# Autodesk Inventor assembly: Shooter Assembly v2
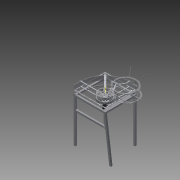
[picture p0: Inventor's stored thumbnail of the model, 180x180]
Saved by Autodesk Inventor 2013 (Build 170138000, 138)
## iProperties
Created: 2013-01-15
Part Number: Shooter Assembly v2
Document SubType Name: Assembly
Designer: actoennies
Mass: 7800.39 g
Surface Area: 25298.1 cm^2
Volume: 4142.24 cm^3
Density: 1.88313 g/cm^3
Author: actoennies
## Documents named in this file (24)
- C:\Users\Moses\Documents\GitHub\frc2013CAD\Launcher\Shooter\Shooter Assembly v2.iam
- C:\Users\Moses\Documents\GitHub\frc2013CAD\Launcher\Shooter\Bearing Mount v1.ipt
- C:\Users\Moses\Documents\GitHub\frc2013CAD\Launcher\Shooter\Outer Rail v1.ipt
- C:\Users\Moses\Documents\GitHub\frc2013CAD\Launcher\Shooter\Runner Rails v2.ipt
- C:\Users\Moses\Documents\GitHub\frc2013CAD\Launcher\Other\8 Plaction Wheel.iam
- C:\Users\Moses\Documents\GitHub\frc2013CAD\Launcher\Shooter\Hub v1.ipt
- C:\Users\Moses\Documents\GitHub\frc2013CAD\Launcher\Shooter\Bearing.ipt
- C:\Users\Moses\Documents\GitHub\frc2013CAD\Launcher\Shooter\Shaft.ipt
- C:\Users\Moses\Documents\GitHub\frc2013CAD\Launcher\Parts\Imported Components\Toughbox Nano 500 key\2mmx2mmx10mm_key.ipt
- C:\Users\Moses\Documents\GitHub\frc2013CAD\Launcher\Shooter\CIM Assembly.iam
- C:\Users\Moses\Documents\GitHub\frc2013CAD\Launcher\Shooter\Flywheel Assembly.iam
- C:\Users\Moses\Documents\GitHub\frc2013CAD\Launcher\Shooter\Shooter Mounter.ipt
- C:\Users\Moses\Documents\GitHub\frc2013CAD\Launcher\Shooter\Bearing Mount 2 v1.ipt
- C:\Users\Moses\Documents\GitHub\frc2013CAD\Launcher\Shooter\Shorter Shaft.ipt
- C:\Users\Moses\Documents\GitHub\frc2013CAD\Launcher\Shooter\Spacer Rube.ipt
- C:\Users\Moses\Documents\GitHub\frc2013CAD\Launcher\Shooter\Tower Angled Mount.ipt
- C:\Users\Moses\Documents\GitHub\frc2013CAD\Launcher\Shooter\Edge Mount.ipt
- C:\Users\Moses\Documents\GitHub\frc2013CAD\Launcher\Shooter\Tower Corner Mount.ipt
- C:\Users\Moses\Documents\GitHub\frc2013CAD\Launcher\Shooter\Square Tube.ipt
- C:\Users\Moses\Documents\GitHub\frc2013CAD\Launcher\Shooter\Flange Bearing Mount Tower.ipt
- C:\Users\Moses\Documents\GitHub\frc2013CAD\Launcher\Shooter\Flange Bearing Mount Tower Mirror.ipt
- C:\Users\Moses\Documents\GitHub\frc2013CAD\Launcher\Shooter\Bearing Mount Top.ipt
- C:\Users\Moses\Documents\GitHub\frc2013CAD\Launcher\Shooter\Square Motor Mount.ipt
- C:\Users\Moses\Documents\GitHub\frc2013CAD\Launcher\Hopper\HopperAssembly42inch_v5.iam
## Components (36 placed, 23 different names)
1. Bearing Mount v1:1 — Insert:12, Insert:13, Insert:14, Insert:15, Insert:19, Angle:1, Insert:26, Insert:27
2. Outer Rail v1:1 — Insert:12, Insert:13, Insert:47, Insert:48, Flush:21
3. Runner Rails v2:1 — Insert:14, Insert:15, Mate:42
4. 8 Plaction Wheel:1 [sub-assembly] — Insert:21, Insert:22, Rotation:1
5. Hub v1:1 — Insert:21, Flush:3, Insert:23
6. Hub v1:2 — Insert:22, Flush:3, Rotation:1, Mate:6
7. Bearing:1 — Mate:3, Insert:49
8. Bearing:2 — Insert:19, Mate:1, Mate:2, Insert:23
9. Shaft:1 — Mate:1, Mate:2, Mate:3, Flush:4, Mate:4, Mate:5, Mate:6, Mate:7, Mate:8, Flush:5
10. 2mmx2mmx10mm_key:1
11. CIM Assembly:1 [sub-assembly] — Flush:4, Mate:4, Mate:5, Angle:1, Mate:9, Mate:10, Mate:11
12. Flywheel Assembly:1 [sub-assembly] — Mate:7, Mate:8, Flush:5, Mate:39
13. Shooter Mounter:1 — Insert:26, Insert:27, Insert:34, Flush:11, Mate:10, Mate:11, Insert:35, Insert:36, Insert:37, Insert:38, Flush:19
14. Spacer Rube:1 — Insert:34, Flush:11
15. Bearing Mount 2 v1:1 — Insert:37, Insert:38, Insert:40
16. Bearing Mount 2 v1:2 — Insert:35, Insert:36, Insert:39
17. Bearing:3 — Insert:40, Flush:13, Mate:14, Mate:15
18. Bearing:4 — Insert:39, Flush:12, Mate:12, Mate:13, Mate:36
19. Shorter Shaft:1 — Flush:12, Mate:12, Mate:13, Mate:37
20. Shorter Shaft:2 — Flush:13, Mate:14, Mate:15, Mate:38
21. Tower Angled Mount:1 — Mate:34, Flush:18, Mate:35, Mate:40, Flush:20
22. Edge Mount:1 — Mate:18, Flush:15, Mate:19, Mate:20, Mate:41
23. Tower Corner Mount:1 — Mate:16, Flush:14, Mate:17
24. Edge Mount:2 — Mate:24, Mate:25, Flush:17, Mate:26, Mate:28
25. Square Tube:1 — Mate:20, Mate:21, Mate:33, Mate:34, Flush:18
26. Square Tube:2 — Mate:16, Flush:14, Mate:17, Mate:18, Flush:15, Mate:19, Mate:21, Mate:22, Mate:23, Flush:16, Insert:41, Insert:42, Flush:19
27. Square Tube:3 — Mate:27, Mate:28, Mate:29, Mate:33, Mate:35, Insert:44, Insert:45
28. Square Tube:4 — Mate:22, Mate:23, Flush:16, Mate:24, Mate:25, Flush:17, Mate:26, Mate:27, Mate:29
29. Flange Bearing Mount Tower:1 — Insert:41, Insert:42, Insert:43
30. Bearing:5 — Insert:43, Mate:36, Mate:37
31. Flange Bearing Mount Tower Mirror:1 — Insert:44, Insert:45, Insert:46
32. Bearing:6 — Insert:46, Mate:38
33. Bearing Mount Top:1 — Insert:47, Insert:48, Insert:49, Mate:39
34. Square Motor Mount:1 — Mate:40, Flush:20, Mate:41
35. HopperAssembly42inch_v5:1 [sub-assembly] — Mate:42, Flush:21
36. Square Motor Mount:2
## Relationships (81: Mate 39, Insert 26, Flush 14, RelateRotation 1, Angle 1)
- Insert:12: Bearing Mount v1:1 ↔ Outer Rail v1:1
- Insert:13: Bearing Mount v1:1 ↔ Outer Rail v1:1
- Insert:14: Bearing Mount v1:1 ↔ Runner Rails v2:1
- Insert:15: Bearing Mount v1:1 ↔ Runner Rails v2:1
- Insert:19: Bearing Mount v1:1 ↔ Bearing:2
- Mate:1: Bearing:2 ↔ Shaft:1
- Mate:2: Bearing:2 ↔ Shaft:1
- Mate:3: Bearing:1 ↔ Shaft:1
- Insert:21: 8 Plaction Wheel:1 ↔ Hub v1:1
- Insert:22: 8 Plaction Wheel:1 ↔ Hub v1:2
- Flush:3: Hub v1:1 ↔ Hub v1:2
- Insert:23 (3.175 mm): Hub v1:1 ↔ Bearing:2
- Rotation:1 [RelateRotation] (1 ul): 8 Plaction Wheel:1 ↔ Hub v1:2
- Flush:4 (6.35 mm): Shaft:1 ↔ CIM Assembly:1
- Mate:4: Shaft:1 ↔ CIM Assembly:1
- Mate:5: Shaft:1 ↔ CIM Assembly:1
- Mate:6: Hub v1:2 ↔ Shaft:1
- Angle:1 (45 deg): Bearing Mount v1:1 ↔ CIM Assembly:1
- Mate:7: Shaft:1 ↔ Flywheel Assembly:1
- Mate:8: Shaft:1 ↔ Flywheel Assembly:1
- Flush:5: Shaft:1 ↔ Flywheel Assembly:1
- Insert:26: Bearing Mount v1:1 ↔ Shooter Mounter:1
- Insert:27: Bearing Mount v1:1 ↔ Shooter Mounter:1
- Insert:34: Shooter Mounter:1 ↔ Spacer Rube:1
- Flush:11: Shooter Mounter:1 ↔ Spacer Rube:1
- Mate:9: CIM Assembly:1
- Mate:10: CIM Assembly:1 ↔ Shooter Mounter:1
- Mate:11: CIM Assembly:1 ↔ Shooter Mounter:1
- Insert:35: Shooter Mounter:1 ↔ Bearing Mount 2 v1:2
- Insert:36: Shooter Mounter:1 ↔ Bearing Mount 2 v1:2
- Insert:37: Shooter Mounter:1 ↔ Bearing Mount 2 v1:1
- Insert:38: Shooter Mounter:1 ↔ Bearing Mount 2 v1:1
- Insert:39: Bearing Mount 2 v1:2 ↔ Bearing:4
- Insert:40: Bearing Mount 2 v1:1 ↔ Bearing:3
- Flush:12 (-25.4 mm): Bearing:4 ↔ Shorter Shaft:1
- Mate:12: Bearing:4 ↔ Shorter Shaft:1
- Mate:13: Bearing:4 ↔ Shorter Shaft:1
- Flush:13 (-25.4 mm): Bearing:3 ↔ Shorter Shaft:2
- Mate:14: Bearing:3 ↔ Shorter Shaft:2
- Mate:15: Bearing:3 ↔ Shorter Shaft:2
- Mate:16: Tower Corner Mount:1 ↔ Square Tube:2
- Flush:14: Tower Corner Mount:1 ↔ Square Tube:2
- Mate:17: Tower Corner Mount:1 ↔ Square Tube:2
- Mate:18: Edge Mount:1 ↔ Square Tube:2
- Flush:15: Edge Mount:1 ↔ Square Tube:2
- Mate:19: Edge Mount:1 ↔ Square Tube:2
- Mate:20: Edge Mount:1 ↔ Square Tube:1
- Mate:21: Square Tube:1 ↔ Square Tube:2
- Mate:22: Square Tube:2 ↔ Square Tube:4
- Mate:23: Square Tube:2 ↔ Square Tube:4
- Flush:16: Square Tube:2 ↔ Square Tube:4
- Mate:24: Edge Mount:2 ↔ Square Tube:4
- Mate:25: Edge Mount:2 ↔ Square Tube:4
- Flush:17: Edge Mount:2 ↔ Square Tube:4
- Mate:26: Edge Mount:2 ↔ Square Tube:4
- Mate:27: Square Tube:3 ↔ Square Tube:4
- Mate:28: Edge Mount:2 ↔ Square Tube:3
- Mate:29: Square Tube:3 ↔ Square Tube:4
- Mate:33: Square Tube:1 ↔ Square Tube:3
- Mate:34: Tower Angled Mount:1 ↔ Square Tube:1
- Flush:18: Tower Angled Mount:1 ↔ Square Tube:1
- Mate:35: Tower Angled Mount:1 ↔ Square Tube:3
- Insert:41: Square Tube:2 ↔ Flange Bearing Mount Tower:1
- Insert:42: Square Tube:2 ↔ Flange Bearing Mount Tower:1
- Insert:43: Flange Bearing Mount Tower:1 ↔ Bearing:5
- Flush:19: Shooter Mounter:1 ↔ Square Tube:2
- Mate:36: Bearing:4 ↔ Bearing:5
- Mate:37: Shorter Shaft:1 ↔ Bearing:5
- Insert:44: Square Tube:3 ↔ Flange Bearing Mount Tower Mirror:1
- Insert:45: Square Tube:3 ↔ Flange Bearing Mount Tower Mirror:1
- Insert:46: Flange Bearing Mount Tower Mirror:1 ↔ Bearing:6
- Mate:38: Shorter Shaft:2 ↔ Bearing:6
- Insert:47: Outer Rail v1:1 ↔ Bearing Mount Top:1
- Insert:48: Outer Rail v1:1 ↔ Bearing Mount Top:1
- Insert:49: Bearing:1 ↔ Bearing Mount Top:1
- Mate:39 (6.35 mm): Flywheel Assembly:1 ↔ Bearing Mount Top:1
- Mate:40: Tower Angled Mount:1 ↔ Square Motor Mount:1
- Flush:20: Tower Angled Mount:1 ↔ Square Motor Mount:1
- Mate:41: Edge Mount:1 ↔ Square Motor Mount:1
- Mate:42: Runner Rails v2:1 ↔ HopperAssembly42inch_v5:1
- Flush:21: Outer Rail v1:1 ↔ HopperAssembly42inch_v5:1
